# Autodesk Inventor assembly: ThinVersaPulley
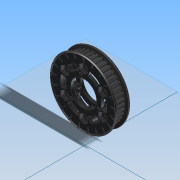
[picture p0: Inventor's stored thumbnail of the model, 180x180]
Saved by Autodesk Inventor 2014 SP2 (Build 180246200, 246)
## iProperties
Created: 2014-06-01
Part Number: ThinVersaPulley
Document SubType Name: Assembly
Designer: dliu
Author: dliu
## Documents named in this file (2)
- C:\Users\dliu\Dropbox\dbhome\electric-longboard\dliu\Pulleys\ThinVersaPulley.iam
- C:\Users\dliu\Dropbox\dbhome\electric-longboard\dliu\Pulleys\217-3199-001 Rev4.ipt
## Components (2 placed, 1 different names)
1. 217-3199-001 Rev4:1 — Insert:1, Insert:2
2. 217-3199-001 Rev4:2 — Insert:1, Insert:2
## Relationships (2: Insert 2)
- Insert:1: 217-3199-001 Rev4:1 ↔ 217-3199-001 Rev4:2
- Insert:2: 217-3199-001 Rev4:1 ↔ 217-3199-001 Rev4:2
